# Autodesk Inventor assembly: 4in traction wheel with 32T Sprockets
Saved by Autodesk Inventor 2013 (Build 170138000, 138)
## iProperties
Created: 2013-05-24
Part Number: 4in traction wheel with 32T Sprockets
Document SubType Name: Assembly
Designer: natsidhu
Author: natsidhu
## Documents named in this file (6)
- \\lmss\STUDENTS\Robotics\CAD Files\COTS Parts\Kit Frame - VexPro\4in traction wheel with 32T Sprockets.iam
- \\lmss\STUDENTS\Robotics\CAD Files\COTS Parts\Wheels\VexPro Traction Wheels\Vex Traction Wheel 4x1.5.iam
- \\lmss\STUDENTS\Robotics\CAD Files\COTS Parts\Bearings - VexPro\Flanged Bearing - 0.5in Round ID x 1.125in OD.ipt
- \\lmss\STUDENTS\Robotics\CAD Files\COTS Parts\Sprockets - VexPro #25\25 Sprocket 32T Vex.ipt
- \\lmss\STUDENTS\Robotics\CAD Files\COTS Parts\Hubs\VersaHub Sprocket Spacer.ipt
- \\lmss\STUDENTS\Robotics\CAD Files\COTS Parts\Fasteners\8-32 BHCS x1000.ipt
## Components (13 placed, 5 different names)
1. Vex Traction Wheel 4x1.5:1 [sub-assembly]
2. Flanged Bearing - 0.5in Round ID x 1.125in OD:1
3. Flanged Bearing - 0.5in Round ID x 1.125in OD:2
4. 25 Sprocket 32T Vex:1
5. 25 Sprocket 32T Vex:2
6. VersaHub Sprocket Spacer:1
7. VersaHub Sprocket Spacer:2
8. 8-32 BHCS x1000:1
9. 8-32 BHCS x1000:2
10. 8-32 BHCS x1000:3
11. 8-32 BHCS x1000:4
12. 8-32 BHCS x1000:5
13. 8-32 BHCS x1000:6
## Component patterns: (3 elements, first: 8-32 BHCS x1000:1 + 8-32 BHCS x1000:2)
## Relationships (19: Mate 17, Insert 2)
- [Mate]: Vex Traction Wheel 4x1.5:1 ↔ Flanged Bearing - 0.5in Round ID x 1.125in OD:1
- [Mate]: Vex Traction Wheel 4x1.5:1 ↔ Flanged Bearing - 0.5in Round ID x 1.125in OD:1
- [Mate]: Vex Traction Wheel 4x1.5:1 ↔ Flanged Bearing - 0.5in Round ID x 1.125in OD:2
- [Mate]: Vex Traction Wheel 4x1.5:1 ↔ Flanged Bearing - 0.5in Round ID x 1.125in OD:2
- [Mate]: Vex Traction Wheel 4x1.5:1 ↔ 25 Sprocket 32T Vex:1
- [Mate]: Vex Traction Wheel 4x1.5:1 ↔ 25 Sprocket 32T Vex:1
- [Mate]: Vex Traction Wheel 4x1.5:1 ↔ VersaHub Sprocket Spacer:1
- [Mate]: Vex Traction Wheel 4x1.5:1 ↔ VersaHub Sprocket Spacer:1
- [Mate]: Vex Traction Wheel 4x1.5:1 ↔ VersaHub Sprocket Spacer:1
- [Mate]: Vex Traction Wheel 4x1.5:1 ↔ VersaHub Sprocket Spacer:1
- [Mate]: 25 Sprocket 32T Vex:1 ↔ VersaHub Sprocket Spacer:1
- [Mate]: Flanged Bearing - 0.5in Round ID x 1.125in OD:2 ↔ VersaHub Sprocket Spacer:2
- [Mate]: Vex Traction Wheel 4x1.5:1 ↔ VersaHub Sprocket Spacer:2
- [Mate]: Vex Traction Wheel 4x1.5:1 ↔ VersaHub Sprocket Spacer:2
- [Mate]: 25 Sprocket 32T Vex:2 ↔ VersaHub Sprocket Spacer:2
- [Mate]: 25 Sprocket 32T Vex:2 ↔ VersaHub Sprocket Spacer:2
- [Insert]: 25 Sprocket 32T Vex:1 ↔ 8-32 BHCS x1000:2
- [Insert]: 25 Sprocket 32T Vex:2 ↔ 8-32 BHCS x1000:1
- [Mate]: 25 Sprocket 32T Vex:2 ↔ VersaHub Sprocket Spacer:2
## Named parameters: d0_d6 = 0 mm, d1_d7 = 0 mm, d2_d8 = 0 mm, d3_d9 = 0 mm, d4_d10 = 0 mm, d5_d11 = 0 mm, d6_d12 = 0 mm, d7_d13 = 0 mm, d8_d14 = 0 mm, d9_d15 = 0 mm, d10_d16 = 0 mm, d11_d17 = 0 mm, d12_d18 = 0 mm, d13_d19 = 120 deg, d14_d20 = 3
